# Autodesk Inventor assembly: AS-070S-0200-10
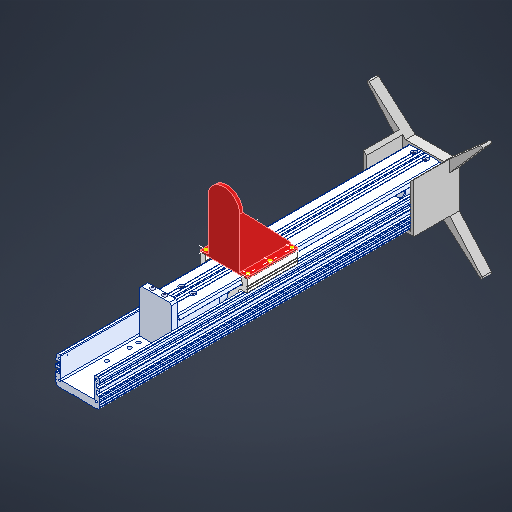
[picture p0: Inventor's stored thumbnail of the model, 512x512]
Saved by Autodesk Inventor 2027 (Build 310192060, 192F)
## iProperties
Created: 2018-09-27
Part Number: AS-070S-0200-10
Description: STEP AP214
Document SubType Name: Assembly
Designer: trtrn
Sending System: SolidWorks 2014
Preprocessor: SwSTEP 2.0
Title: AS-070S-0200-10.STEP
Author: user
Revision Number: ANY
## Documents named in this file (8)
- G:\My Drive\Project\GLUE01\Cad\PA1\AS-070S-0200-10.iam
- G:\My Drive\Project\GLUE01\Cad\PA1\AS-070S-0200 MAIN BASE.ipt
- G:\My Drive\Project\GLUE01\Cad\PA1\TRUSS M4x10L-2_Ç¥ÁØ.ipt
- G:\My Drive\Project\GLUE01\Cad\PA1\WRENCH BOLT M4x12L_Ç¥ÁØ.ipt
- G:\My Drive\Project\GLUE01\Cad\PA1\AS-070-SLIDER.ipt
- G:\My Drive\Project\GLUE01\Cad\PA1\Dam1.ipt
- G:\My Drive\Project\GLUE01\Cad\PA1\Syringe_100ml\Syringe_100ml.ipt
- G:\My Drive\Project\GLUE01\Cad\PA1\KeChan.ipt
## Components (15 placed, 15 different names)
1. AS-070S-0200 MAIN BASE_1 — Mate:1, Angle:1, Mate:20, Mate:21, Mate:22, Mate:23, Mate:32
2. WRENCH BOLT M4x12L_Ç¥ÁØ_5 — Mate:25, Mate:30
3. TRUSS M4x10L-2_Ç¥ÁØ_6
4. TRUSS M4x10L-2_Ç¥ÁØ_7
5. WRENCH BOLT M4x12L_Ç¥ÁØ_8 — Mate:26, Mate:28
6. WRENCH BOLT M4x12L_Ç¥ÁØ_9 — Mate:27, Mate:29
7. WRENCH BOLT M4x12L_Ç¥ÁØ_10 — Mate:24, Mate:31
8. TRUSS M4x10L-2_Ç¥ÁØ_11
9. TRUSS M4x10L-2_Ç¥ÁØ_12
10. TRUSS M4x10L-2_Ç¥ÁØ_13
11. TRUSS M4x10L-2_Ç¥ÁØ_14
12. AS-070-SLIDER_21 — Mate:1, Angle:1, Flush:1, Flush:2, Mate:2, Mate:32
13. Dam1:1 — Flush:1, Flush:2, Mate:2, Mate:16, Mate:17, Mate:18, Mate:19
14. Syringe_100ml:1 — Mate:18, Mate:19
15. KeChan:1 — Mate:20, Mate:21, Mate:22, Mate:23, Mate:24, Mate:25, Mate:26, Mate:27, Mate:28, Mate:29, Mate:30, Mate:31
## Relationships (22: Mate 19, Flush 2, Angle 1)
- Mate:1: AS-070S-0200 MAIN BASE_1 ↔ AS-070-SLIDER_21
- Angle:1 (0 deg): AS-070S-0200 MAIN BASE_1 ↔ AS-070-SLIDER_21
- Flush:1: AS-070-SLIDER_21 ↔ Dam1:1
- Flush:2: AS-070-SLIDER_21 ↔ Dam1:1
- Mate:2: AS-070-SLIDER_21 ↔ Dam1:1
- Mate:16: Dam1:1
- Mate:17: Dam1:1
- Mate:18: Dam1:1 ↔ Syringe_100ml:1
- Mate:19: Dam1:1 ↔ Syringe_100ml:1
- Mate:20: AS-070S-0200 MAIN BASE_1 ↔ KeChan:1
- Mate:21: AS-070S-0200 MAIN BASE_1 ↔ KeChan:1
- Mate:22: AS-070S-0200 MAIN BASE_1 ↔ KeChan:1
- Mate:23: AS-070S-0200 MAIN BASE_1 ↔ KeChan:1
- Mate:24: WRENCH BOLT M4x12L_Ç¥ÁØ_10 ↔ KeChan:1
- Mate:25: WRENCH BOLT M4x12L_Ç¥ÁØ_5 ↔ KeChan:1
- Mate:26: WRENCH BOLT M4x12L_Ç¥ÁØ_8 ↔ KeChan:1
- Mate:27: WRENCH BOLT M4x12L_Ç¥ÁØ_9 ↔ KeChan:1
- Mate:28: WRENCH BOLT M4x12L_Ç¥ÁØ_8 ↔ KeChan:1
- Mate:29: WRENCH BOLT M4x12L_Ç¥ÁØ_9 ↔ KeChan:1
- Mate:30: WRENCH BOLT M4x12L_Ç¥ÁØ_5 ↔ KeChan:1
- Mate:31: WRENCH BOLT M4x12L_Ç¥ÁØ_10 ↔ KeChan:1
- Mate:32: AS-070S-0200 MAIN BASE_1 ↔ AS-070-SLIDER_21
